# Autodesk Inventor assembly: anschluss_daten_MIR
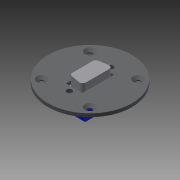
[picture p0: Inventor's stored thumbnail of the model, 180x180]
Saved by Autodesk Inventor 2015 (Build 190159000, 159)
## iProperties
Created: 2018-04-03
Part Number: anschluss_daten_MIR
Document SubType Name: Assembly
Designer: wepet
Author: wepet
## Documents named in this file (3)
- C:\workspace\robosax\licht\Zusatzelemente\anschluss_daten_MIR.iam
- C:\workspace\robosax\licht\Zusatzelemente\anschluss_daten_1_MIR.ipt
- C:\workspace\robosax\licht\Zusatzelemente\anschluss_daten_2_MIR.ipt
## Components (2 placed, 2 different names)
1. anschluss_daten_1_MIR:1 — Drehbar:2, Drehbar:1
2. anschluss_daten_2_MIR:1 — Fluchtend:1, Passend:2, Drehbar:2, Drehbar:1
## Relationships (4: RevoluteJoint 2, Flush 1, Mate 1)
- Fluchtend:1 [Flush] (-15.405 mm): anschluss_daten_2_MIR:1
- Passend:2 [Mate] (-4.18 mm): anschluss_daten_2_MIR:1
- Drehbar:2 [RevoluteJoint] (-3 mm): anschluss_daten_1_MIR:1 ↔ anschluss_daten_2_MIR:1
- Drehbar:1 [RevoluteJoint] (-3 mm): anschluss_daten_1_MIR:1 ↔ anschluss_daten_2_MIR:1
